# Autodesk Inventor assembly: 10-SUSP-ARM
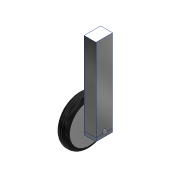
[picture p0: Inventor's stored thumbnail of the model, 180x180]
Saved by Autodesk Inventor 2018 (Build 220112000, 112)
## iProperties
Created: 2017-07-19
Part Number: 10-SUSP-ARM
Document SubType Name: Assembly
Designer: feesmrt
Author: feesmrt
## Documents named in this file (4)
- C:\Users\feesmrt\Documents\NRBDL\Inventor-NRBDL\10-SUSP\10-SUSP-ARM.iam
- C:\Users\feesmrt\Documents\NRBDL\Inventor-NRBDL\10-SUSP\10-001-ACTR.ipt
- C:\Users\feesmrt\Documents\NRBDL\Inventor-NRBDL\10-SUSP\10-002-ARM.ipt
- C:\Users\feesmrt\Documents\NRBDL\Inventor-NRBDL\10-SUSP\10-003-ARM-CAP.ipt
## Components (3 placed, 3 different names)
1. 10-002-ARM:1 — Mate:1, Angle:1, Mate:2, Mate:3, Flush:1, Flush:2
2. 10-001-ACTR:1 — Mate:1, Angle:1, Mate:2
3. 10-003-ARM-CAP:1 — Mate:3, Flush:1, Flush:2
## Relationships (6: Mate 3, Flush 2, Angle 1)
- Mate:1: 10-002-ARM:1 ↔ 10-001-ACTR:1
- Angle:1 (0 deg): 10-002-ARM:1 ↔ 10-001-ACTR:1
- Mate:2 (0.5 mm): 10-002-ARM:1 ↔ 10-001-ACTR:1
- Mate:3: 10-002-ARM:1 ↔ 10-003-ARM-CAP:1
- Flush:1: 10-002-ARM:1 ↔ 10-003-ARM-CAP:1
- Flush:2: 10-002-ARM:1 ↔ 10-003-ARM-CAP:1
